# Autodesk Inventor assembly: bearing_nrt_260_b_0
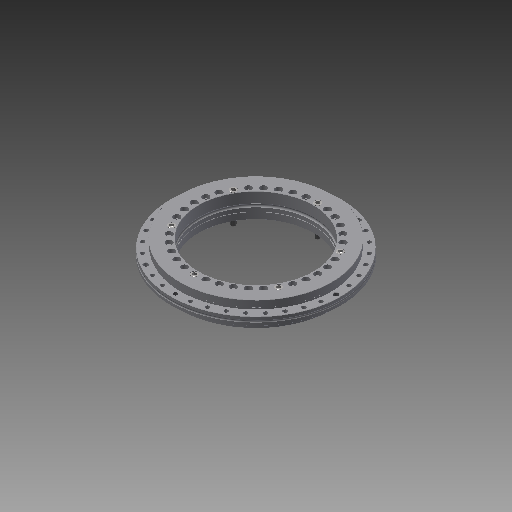
[picture p0: Inventor's stored thumbnail of the model, 512x512]
Saved by Autodesk Inventor 2019 (Build 230136000, 136)
## iProperties
Company: TraceParts S.A.
Created: 2019-11-22
Part Number: bearing_nrt_260_b_0
Checked By: TraceParts S.A.
Catalog Web Link: www.traceparts.com
Document SubType Name: Assembly
Designer: TraceParts
Mass: 2694.67 g
Surface Area: 5068.65 cm^2
Volume: 2433.07 cm^3
Density: 1.10752 g/cm^3
REFERENCE: NRT 260 B
SUPPLIER: SKF
MASS: 18.2 kg
DESIGN: Axial-radial cylindrical roller bearings, super-precision, Bore Ø 260 mm
TraceParts.PartVersion: 1.0.4
TraceParts.PartNumber: 33-12092018-072853
TraceParts.PartLanguage: en
TraceParts.InstanceId: 33-12092018-0728537K8Q807F6YJ5CG6RTO5S8QPP6
TraceParts.PartTitle: Axial-radial cylindrical roller bearings, super-precision
TRACEPARTS: TRACEPARTS
TraceParts.ClassPath: SKF:33-12092018-072853
TraceParts.PartStatus: Published
Author: TraceParts
## Documents named in this file (5)
- D:\Downloads\95961009-9-bearing_nrt_260_b_0\bearing_nrt_260_b_0.iam
- D:\Downloads\95961009-9-bearing_nrt_260_b_0\bearing_nrt_260_b_0_01.ipt
- D:\Downloads\95961009-9-bearing_nrt_260_b_0\bearing_nrt_260_b_0_02.ipt
- D:\Downloads\95961009-9-bearing_nrt_260_b_0\bearing_nrt_260_b_0_03.ipt
- D:\Documents\Inventor\Content Center Files\R2019\en-US\AS 1420\AS 1420 - 1973 - M10 x 60.ipt
## Components (9 placed, 4 different names)
1. bearing_nrt_260_b_0_01:1 — Mate:3, Mate:4, Mate:5, Mate:6, Mate:7, Mate:8, Mate:9, Mate:10, Mate:11, Mate:12, Mate:13, Mate:14, Mate:15, Mate:16, Mate:17, Mate:18, Mate:19
2. bearing_nrt_260_b_0_02:1 — Mate:2, Mate:6
3. bearing_nrt_260_b_0_03:1 — Mate:1, Mate:5, Mate:7
4. AS 1420 - Metric M10 x 60:1 — Mate:8, Mate:14
5. AS 1420 - Metric M10 x 60:2 — Mate:9, Mate:17
6. AS 1420 - Metric M10 x 60:3 — Mate:10, Mate:15
7. AS 1420 - Metric M10 x 60:4 — Mate:11, Mate:18
8. AS 1420 - Metric M10 x 60:5 — Mate:13, Mate:16
9. AS 1420 - Metric M10 x 60:6 — Mate:12, Mate:19
## Relationships (19: Mate 19)
- Mate:1: bearing_nrt_260_b_0_03:1
- Mate:2: bearing_nrt_260_b_0_02:1
- Mate:3: bearing_nrt_260_b_0_01:1
- Mate:4: bearing_nrt_260_b_0_01:1
- Mate:5: bearing_nrt_260_b_0_01:1 ↔ bearing_nrt_260_b_0_03:1
- Mate:6: bearing_nrt_260_b_0_01:1 ↔ bearing_nrt_260_b_0_02:1
- Mate:7: bearing_nrt_260_b_0_01:1 ↔ bearing_nrt_260_b_0_03:1
- Mate:8: bearing_nrt_260_b_0_01:1 ↔ AS 1420 - Metric M10 x 60:1
- Mate:9: bearing_nrt_260_b_0_01:1 ↔ AS 1420 - Metric M10 x 60:2
- Mate:10: bearing_nrt_260_b_0_01:1 ↔ AS 1420 - Metric M10 x 60:3
- Mate:11: bearing_nrt_260_b_0_01:1 ↔ AS 1420 - Metric M10 x 60:4
- Mate:12: bearing_nrt_260_b_0_01:1 ↔ AS 1420 - Metric M10 x 60:6
- Mate:13: bearing_nrt_260_b_0_01:1 ↔ AS 1420 - Metric M10 x 60:5
- Mate:14 (-10 mm): bearing_nrt_260_b_0_01:1 ↔ AS 1420 - Metric M10 x 60:1
- Mate:15 (-10 mm): bearing_nrt_260_b_0_01:1 ↔ AS 1420 - Metric M10 x 60:3
- Mate:16 (-10 mm): bearing_nrt_260_b_0_01:1 ↔ AS 1420 - Metric M10 x 60:5
- Mate:17 (-10 mm): bearing_nrt_260_b_0_01:1 ↔ AS 1420 - Metric M10 x 60:2
- Mate:18 (-10 mm): bearing_nrt_260_b_0_01:1 ↔ AS 1420 - Metric M10 x 60:4
- Mate:19 (-10 mm): bearing_nrt_260_b_0_01:1 ↔ AS 1420 - Metric M10 x 60:6
